# Autodesk Inventor assembly: Drone_wing
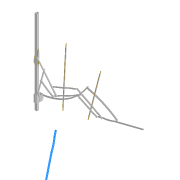
[picture p0: Inventor's stored thumbnail of the model, 180x180]
Saved by Autodesk Inventor 2022 (Build 260153000, 153)
## iProperties
Created: 2022-05-03
Part Number: Drone_wing
Document SubType Name: Assembly
Designer: dell
Author: dell
## Documents named in this file (18)
- D:\xxxx\Uni\Part IV\MECHENG_700\Part_IV_project_CAD\Bird_skeleton_prototypes\Wing_drone_V1\Drone_wing.iam
- D:\xxxx\Uni\Part IV\MECHENG_700\Part_IV_project_CAD\Bird_skeleton_prototypes\Wing_drone_V1\Square_tube_connector.ipt
- D:\xxxx\Uni\Part IV\MECHENG_700\Part_IV_project_CAD\Bird_skeleton_prototypes\Wing_drone_V1\Square_tube_arm.ipt
- D:\xxxx\Uni\Part IV\MECHENG_700\Part_IV_project_CAD\Bird_skeleton_prototypes\Wing_drone_V1\Drone_wing_skeleton_V11\Rail.ipt
- D:\xxxx\Uni\Part IV\MECHENG_700\Part_IV_project_CAD\Bird_skeleton_prototypes\Wing_drone_V1\Drone_wing_skeleton_V11\Part_2.ipt
- D:\xxxx\Uni\Part IV\MECHENG_700\Part_IV_project_CAD\Bird_skeleton_prototypes\Wing_drone_V1\Drone_wing_skeleton_V11\Part_3.ipt
- D:\xxxx\Uni\Part IV\MECHENG_700\Part_IV_project_CAD\Bird_skeleton_prototypes\Wing_drone_V1\Drone_wing_skeleton_V11\Part_4.ipt
- D:\xxxx\Uni\Part IV\MECHENG_700\Part_IV_project_CAD\Bird_skeleton_prototypes\Wing_drone_V1\Drone_wing_skeleton_V11\Part_16.ipt
- D:\xxxx\Uni\Part IV\MECHENG_700\Part_IV_project_CAD\Bird_skeleton_prototypes\Wing_drone_V1\Drone_wing_skeleton_V11\Part_5.ipt
- D:\xxxx\Uni\Part IV\MECHENG_700\Part_IV_project_CAD\Bird_skeleton_prototypes\Wing_drone_V1\Drone_wing_skeleton_V11\Part_7.ipt
- D:\xxxx\Uni\Part IV\MECHENG_700\Part_IV_project_CAD\Bird_skeleton_prototypes\Wing_drone_V1\Drone_wing_skeleton_V11\Part_9.ipt
- D:\xxxx\Uni\Part IV\MECHENG_700\Part_IV_project_CAD\Bird_skeleton_prototypes\Wing_drone_V1\Drone_wing_skeleton_V11\Part_10.ipt
- D:\xxxx\Uni\Part IV\MECHENG_700\Part_IV_project_CAD\Bird_skeleton_prototypes\Wing_drone_V1\Drone_wing_skeleton_V11\Part_12.ipt
- D:\xxxx\Uni\Part IV\MECHENG_700\Part_IV_project_CAD\Bird_skeleton_prototypes\Wing_drone_V1\Drone_wing_skeleton_V11\Part_14.ipt
- D:\xxxx\Uni\Part IV\MECHENG_700\Part_IV_project_CAD\Bird_skeleton_prototypes\Wing_drone_V1\Drone_wing_skeleton_V11\Part_11.ipt
- D:\xxxx\Uni\Part IV\MECHENG_700\Part_IV_project_CAD\Bird_skeleton_prototypes\Wing_drone_V1\Drone_wing_skeleton_V11\Part_8.ipt
- D:\xxxx\Uni\Part IV\MECHENG_700\Part_IV_project_CAD\Bird_skeleton_prototypes\Wing_drone_V1\Motor_mount.ipt
- D:\xxxx\Uni\Part IV\MECHENG_700\Part_IV_project_CAD\Bird_skeleton_prototypes\Wing_drone_V1\XM430.iam
## Components (18 placed, 17 different names)
1. Square_tube_connector:1 — Mate:1, Mate:2, Mate:3, Mate:4, Mate:5, Mate:6, Mate:9, Flush:9
2. Square_tube_arm:1 — Mate:1, Mate:2, Mate:3, Mate:8, Flush:5
3. Square_tube_arm:2 — Mate:4, Mate:5, Mate:6, Mate:52, Mate:53
4. Rail:1 — Mate:8, Mate:9, Mate:16, Flush:5
5. Part_2:1 — Mate:12, Mate:15, Mate:17, Mate:18, Mate:57, Mate:58
6. Part_3:1 — Mate:12, Mate:15, Mate:16, Mate:21, Mate:22, Mate:23
7. Part_4:1 — Mate:17, Mate:18, Mate:19, Mate:20
8. Part_16:1 — Mate:19, Mate:20, Mate:21, Mate:24, Mate:26, Mate:27, Mate:28, Mate:41, Mate:42
9. Part_5:1 — Mate:22, Mate:23, Mate:25, Mate:44
10. Part_7:1 — Mate:24, Mate:25, Mate:26, Mate:30, Mate:31, Mate:45
11. Part_9:1 — Mate:27, Mate:28, Mate:29, Mate:40, Mate:43
12. Part_10:1 — Mate:29, Mate:30, Mate:31, Mate:32, Mate:60
13. Part_12:1 — Mate:32, Mate:50, Mate:51, Mate:60
14. Part_11:1 — Mate:40, Mate:43, Mate:45
15. Part_8:1 — Mate:41, Mate:42, Mate:44
16. Part_14:1 — Mate:50, Mate:51, Mate:63
17. Motor_mount:1 — Mate:52, Mate:53, Flush:9, Mate:57, Mate:58, Mate:61, Mate:62
18. XM430:4 [sub-assembly] — Mate:61, Mate:62, Mate:63
## Relationships (45: Mate 43, Flush 2)
- Mate:1 (0.05 mm): Square_tube_connector:1 ↔ Square_tube_arm:1
- Mate:2 (0.05 mm): Square_tube_connector:1 ↔ Square_tube_arm:1
- Mate:3: Square_tube_connector:1 ↔ Square_tube_arm:1
- Mate:4 (0.05 mm): Square_tube_connector:1 ↔ Square_tube_arm:2
- Mate:5 (0.05 mm): Square_tube_connector:1 ↔ Square_tube_arm:2
- Mate:6: Square_tube_connector:1 ↔ Square_tube_arm:2
- Mate:8: Square_tube_arm:1 ↔ Rail:1
- Mate:9 (15 mm): Square_tube_connector:1 ↔ Rail:1
- Mate:12: Part_2:1 ↔ Part_3:1
- Mate:15: Part_2:1 ↔ Part_3:1
- Mate:16: Rail:1 ↔ Part_3:1
- Mate:17: Part_2:1 ↔ Part_4:1
- Mate:18: Part_2:1 ↔ Part_4:1
- Flush:5: Square_tube_arm:1 ↔ Rail:1
- Mate:19: Part_4:1 ↔ Part_16:1
- Mate:20: Part_4:1 ↔ Part_16:1
- Mate:21: Part_3:1 ↔ Part_16:1
- Mate:22: Part_3:1 ↔ Part_5:1
- Mate:23: Part_3:1 ↔ Part_5:1
- Mate:24: Part_16:1 ↔ Part_7:1
- Mate:25: Part_5:1 ↔ Part_7:1
- Mate:26: Part_16:1 ↔ Part_7:1
- Mate:27: Part_16:1 ↔ Part_9:1
- Mate:28: Part_16:1 ↔ Part_9:1
- Mate:29: Part_9:1 ↔ Part_10:1
- Mate:30: Part_7:1 ↔ Part_10:1
- Mate:31: Part_7:1 ↔ Part_10:1
- Mate:32: Part_10:1 ↔ Part_12:1
- Mate:40: Part_9:1 ↔ Part_11:1
- Mate:41: Part_16:1 ↔ Part_8:1
- Mate:42: Part_16:1 ↔ Part_8:1
- Mate:43: Part_9:1 ↔ Part_11:1
- Mate:44: Part_5:1 ↔ Part_8:1
- Mate:45: Part_7:1 ↔ Part_11:1
- Mate:50: Part_12:1 ↔ Part_14:1
- Mate:51: Part_12:1 ↔ Part_14:1
- Mate:52: Square_tube_arm:2 ↔ Motor_mount:1
- Mate:53: Square_tube_arm:2 ↔ Motor_mount:1
- Flush:9 (270 mm): Square_tube_connector:1 ↔ Motor_mount:1
- Mate:57: Part_2:1 ↔ Motor_mount:1
- Mate:58: Part_2:1 ↔ Motor_mount:1
- Mate:60: Part_10:1 ↔ Part_12:1
- Mate:61: Motor_mount:1 ↔ XM430:4
- Mate:62: Motor_mount:1 ↔ XM430:4
- Mate:63: Part_14:1 ↔ XM430:4
